# Autodesk Inventor assembly: 12
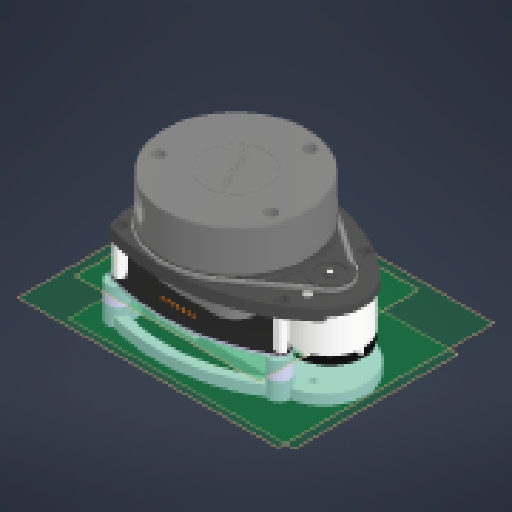
[picture p0: Inventor's stored thumbnail of the model, 512x512]
Saved by Autodesk Inventor 2027 (Build 310192000, 192)
## iProperties
Created: 2023-09-21
Part Number: 12
Description: STEP AP214
Document SubType Name: Assembly
Designer: uchiha
Sending System: SolidWorks 2020
Preprocessor: SwSTEP 2.0
Title: 12.STEP
Revision Number: ANY
## Documents named in this file (3)
- C:\Users\uchiha\Desktop\New folder\designdj\parts\parts\rplidar-a1-holder-1.snapshot.2\12\12.iam
- C:\Users\uchiha\Desktop\New folder\designdj\parts\parts\rplidar-a1-holder-1.snapshot.2\12\RP-lidar-A1.igs.iam
- C:\Users\uchiha\Desktop\New folder\designdj\parts\parts\rplidar-a1-holder-1.snapshot.2\12\Part22.ipt
## Components (2 placed, 2 different names)
1. RP-lidar-A1.igs_1 [sub-assembly] — Symmetry:1
2. Part22_2 — Symmetry:1, Flush:1
## Relationships (2: Symmetry 1, Flush 1)
- Symmetry:1: RP-lidar-A1.igs_1 ↔ Part22_2
- Flush:1: Part22_2
